# Autodesk Inventor assembly: ForkMountWith6inchBevelGear
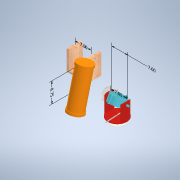
[picture p0: Inventor's stored thumbnail of the model, 180x180]
Saved by Autodesk Inventor 2021.1 (Build 251245010, 245A)
## iProperties
Created: 2020-06-16
Part Number: ForkMountWith6inchBevelGear
Document SubType Name: Assembly
Designer: robst
Author: robst
## Documents named in this file (10)
- C:\git\CAD-Development\robSteele\ShapeWays\TelescopeProjects\TelescopeMount\ForkMountWith6inchBevelGear.iam
- C:\git\CAD-Development\robSteele\ShapeWays\TelescopeProjects\TelescopeMount\topOfRaBase.ipt
- C:\git\CAD-Development\robSteele\ShapeWays\TelescopeProjects\TelescopeMount\baseForBevelGearMount.ipt
- C:\git\CAD-Development\robSteele\ShapeWays\TelescopeProjects\TelescopeMount\10x3_8-keyedDriveShaft.ipt
- C:\git\CAD-Development\robSteele\ShapeWays\TelescopeProjects\TelescopeMount\raHandController.ipt
- C:\git\CAD-Development\robSteele\ShapeWays\TelescopeProjects\TelescopeMount\telescopeTube.ipt
- C:\git\CAD-Development\robSteele\ShapeWays\TelescopeProjects\TelescopeMount\tubeBracket.ipt
- C:\git\CAD-Development\robSteele\ShapeWays\TelescopeProjects\TelescopeMount\ForkMountWith6inchBevelGear\Design Accelerator\Bevel Gears1.iam
- C:\git\CAD-Development\robSteele\ShapeWays\TelescopeProjects\TelescopeMount\ForkMountWith6inchBevelGear\oneHalfForkSupport.ipt
- C:\git\CAD-Development\robSteele\ShapeWays\TelescopeProjects\TelescopeMount\ForkMountWith6inchBevelGear\Design Accelerator\Worm Gears2.iam
## Components (11 placed, 9 different names)
1. topOfRaBase:1 — Insert:3, Insert:26, Mate:6
2. baseForBevelGearMount:1 — Insert:3
3. 10x3_8-keyedDriveShaft:1 — Insert:5
4. raHandController:1 — Insert:5
5. telescopeTube:1
6. tubeBracket:1 — Flush:1, Flush:2, Mate:5
7. tubeBracket:2 — Flush:1, Insert:26, Flush:2
8. Bevel Gears:1 [sub-assembly] — Mate:6
9. oneHalfForkSupport:1 — Mate:2, Flush:3, Flush:4
10. oneHalfForkSupport:2 — Mate:2, Flush:3, Flush:4
11. Worm Gears:2 [sub-assembly] — Mate:5
## Relationships (10: Flush 4, Insert 3, Mate 3)
- Insert:3: topOfRaBase:1 ↔ baseForBevelGearMount:1
- Insert:5: 10x3_8-keyedDriveShaft:1 ↔ raHandController:1
- Flush:1: tubeBracket:1 ↔ tubeBracket:2
- Insert:26 (-38.1 mm): topOfRaBase:1 ↔ tubeBracket:2
- Flush:2: tubeBracket:1 ↔ tubeBracket:2
- Mate:2: oneHalfForkSupport:1 ↔ oneHalfForkSupport:2
- Flush:3: oneHalfForkSupport:1 ↔ oneHalfForkSupport:2
- Flush:4: oneHalfForkSupport:1 ↔ oneHalfForkSupport:2
- Mate:5: tubeBracket:1 ↔ Worm Gears:2
- Mate:6: topOfRaBase:1 ↔ Bevel Gears:1
